# Autodesk Inventor assembly: prototype
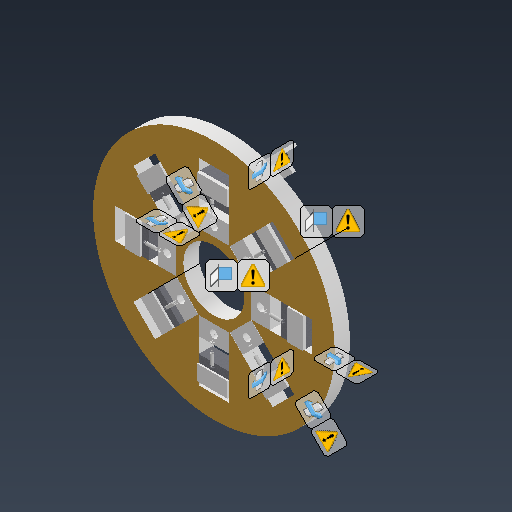
[picture p0: Inventor's stored thumbnail of the model, 512x512]
Saved by Autodesk Inventor 2025.3 (Build 293356000, 356)
## iProperties
Created: 2025-12-15
Part Number: prototype
Document SubType Name: Assembly
Designer: 陳泓任
Author: 陳泓任
## Documents named in this file (6)
- C:\Users\Ou918\ECB_project\CAD\prototype.iam
- C:\Users\Ou918\ECB_project\CAD\yoke.ipt
- C:\Users\Ou918\ECB_project\CAD\slider.ipt
- C:\Users\Ou918\ECB_project\CAD\magnet.ipt
- C:\Users\Ou918\ECB_project\CAD\spring_connect.ipt
- C:\Users\Ou918\ECB_project\CAD\AUA2-10.ipt
## Components (33 placed, 5 different names)
1. yoke:1 — 滑塊:1, 滑塊:2, 滑塊:3, 滑塊:4, 滑塊:5, 滑塊:6, 滑塊:7, 滑塊:8, 旋轉:1, 貼合:21, 貼合:22, 貼合:23, 貼合:24, 貼合:25, 貼合:26, 貼合:27, 貼合:28, 旋轉:2, 旋轉:3, 旋轉:4, 旋轉:5, 旋轉:6, 旋轉:7, 旋轉:8
2. slider:1 — 滑塊:1, 貼合:1, 貼合:2, 齊平:5, 貼合:30
3. slider:2 — 貼合:4, 齊平:1, 貼合:5, 滑塊:2, 貼合:31
4. slider:3 — 貼合:6, 貼合:7, 齊平:2, 滑塊:3, 貼合:33
5. slider:4 — 貼合:8, 貼合:9, 齊平:3, 滑塊:4, 貼合:32
6. slider:5 — 貼合:10, 齊平:4, 貼合:11, 滑塊:5, 貼合:34
7. slider:6 — 滑塊:6, 貼合:12, 貼合:13, 齊平:15
8. slider:7 — 滑塊:7, 貼合:15, 齊平:17, 貼合:17
9. slider:8 — 滑塊:8, 貼合:18, 齊平:20, 貼合:20, 貼合:29
10. magnet:1 — 貼合:1, 貼合:2, 齊平:5
11. magnet:2 — 貼合:4, 齊平:1, 貼合:5
12. magnet:3 — 貼合:6, 貼合:7, 齊平:2
13. magnet:4 — 貼合:8, 貼合:9, 齊平:3
14. magnet:5 — 貼合:10, 齊平:4, 貼合:11
15. magnet:6 — 貼合:12, 貼合:13, 齊平:15
16. magnet:7 — 貼合:15, 齊平:17, 貼合:17
17. magnet:8 — 貼合:18, 齊平:20, 貼合:20
18. spring_connect:1 — 旋轉:1, 貼合:21
19. spring_connect:2 — 貼合:22, 旋轉:2
20. spring_connect:3 — 貼合:23, 旋轉:3
21. spring_connect:4 — 貼合:24, 旋轉:4
22. spring_connect:5 — 貼合:25, 旋轉:6, 貼合:35
23. spring_connect:6 — 貼合:26, 旋轉:5
24. spring_connect:7 — 貼合:27, 旋轉:7, 貼合:36
25. spring_connect:8 — 貼合:28, 旋轉:8
26. AUA2-10:1 — 貼合:29
27. AUA2-10:2 — 貼合:30
28. AUA2-10:3 — 貼合:31
29. AUA2-10:4 — 貼合:36
30. AUA2-10:5 — 貼合:35
31. AUA2-10:6 — 貼合:34
32. AUA2-10:7 — 貼合:32
33. AUA2-10:8 — 貼合:33
## Relationships (56: Mate 32, TranslationJoint 8, Flush 8, RevoluteJoint 8)
- 滑塊:1 [TranslationJoint]: yoke:1 ↔ slider:1
- 貼合:1 [Mate]: slider:1 ↔ magnet:1
- 貼合:2 [Mate]: slider:1 ↔ magnet:1
- 齊平:5 [Flush]: slider:1 ↔ magnet:1
- 貼合:4 [Mate]: slider:2 ↔ magnet:2
- 齊平:1 [Flush]: slider:2 ↔ magnet:2
- 貼合:5 [Mate]: slider:2 ↔ magnet:2
- 貼合:6 [Mate]: slider:3 ↔ magnet:3
- 貼合:7 [Mate]: slider:3 ↔ magnet:3
- 齊平:2 [Flush]: slider:3 ↔ magnet:3
- 貼合:8 [Mate]: slider:4 ↔ magnet:4
- 貼合:9 [Mate]: slider:4 ↔ magnet:4
- 齊平:3 [Flush]: slider:4 ↔ magnet:4
- 貼合:10 [Mate]: slider:5 ↔ magnet:5
- 齊平:4 [Flush]: slider:5 ↔ magnet:5
- 貼合:11 [Mate]: slider:5 ↔ magnet:5
- 滑塊:2 [TranslationJoint]: yoke:1 ↔ slider:2
- 滑塊:3 [TranslationJoint]: yoke:1 ↔ slider:3
- 滑塊:4 [TranslationJoint]: yoke:1 ↔ slider:4
- 滑塊:5 [TranslationJoint]: yoke:1 ↔ slider:5
- 滑塊:6 [TranslationJoint]: yoke:1 ↔ slider:6
- 滑塊:7 [TranslationJoint]: yoke:1 ↔ slider:7
- 滑塊:8 [TranslationJoint]: yoke:1 ↔ slider:8
- 貼合:12 [Mate]: slider:6 ↔ magnet:6
- 貼合:13 [Mate]: slider:6 ↔ magnet:6
- 齊平:15 [Flush]: slider:6 ↔ magnet:6
- 貼合:15 [Mate]: slider:7 ↔ magnet:7
- 齊平:17 [Flush]: slider:7 ↔ magnet:7
- 貼合:17 [Mate]: slider:7 ↔ magnet:7
- 貼合:18 [Mate]: slider:8 ↔ magnet:8
- 齊平:20 [Flush]: slider:8 ↔ magnet:8
- 貼合:20 [Mate]: slider:8 ↔ magnet:8
- 旋轉:1 [RevoluteJoint]: yoke:1 ↔ spring_connect:1
- 貼合:21 [Mate]: yoke:1 ↔ spring_connect:1
- 貼合:22 [Mate]: yoke:1 ↔ spring_connect:2
- 貼合:23 [Mate]: yoke:1 ↔ spring_connect:3
- 貼合:24 [Mate]: yoke:1 ↔ spring_connect:4
- 貼合:25 [Mate]: yoke:1 ↔ spring_connect:5
- 貼合:26 [Mate]: yoke:1 ↔ spring_connect:6
- 貼合:27 [Mate]: yoke:1 ↔ spring_connect:7
- 貼合:28 [Mate]: yoke:1 ↔ spring_connect:8
- 旋轉:2 [RevoluteJoint]: yoke:1 ↔ spring_connect:2
- 旋轉:3 [RevoluteJoint]: yoke:1 ↔ spring_connect:3
- 旋轉:4 [RevoluteJoint]: yoke:1 ↔ spring_connect:4
- 旋轉:5 [RevoluteJoint]: yoke:1 ↔ spring_connect:6
- 旋轉:6 [RevoluteJoint]: yoke:1 ↔ spring_connect:5
- 旋轉:7 [RevoluteJoint]: yoke:1 ↔ spring_connect:7
- 旋轉:8 [RevoluteJoint]: yoke:1 ↔ spring_connect:8
- 貼合:29 [Mate]: slider:8 ↔ AUA2-10:1
- 貼合:30 [Mate]: slider:1 ↔ AUA2-10:2
- 貼合:31 [Mate]: slider:2 ↔ AUA2-10:3
- 貼合:32 [Mate]: slider:4 ↔ AUA2-10:7
- 貼合:33 [Mate]: slider:3 ↔ AUA2-10:8
- 貼合:34 [Mate]: slider:5 ↔ AUA2-10:6
- 貼合:35 [Mate]: spring_connect:5 ↔ AUA2-10:5
- 貼合:36 [Mate]: spring_connect:7 ↔ AUA2-10:4
